# Autodesk Inventor assembly: ThrustBearingAssembly
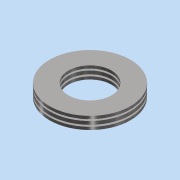
[picture p0: Inventor's stored thumbnail of the model, 180x180]
Saved by Autodesk Inventor 2017 (Build 210142000, 142)
## iProperties
Created: 2016-11-28
Part Number: ThrustBearingAssembly
Document SubType Name: Assembly
Designer: techn
Author: techn
## Documents named in this file (3)
- D:\OneDrive\Documents\Other Projects\Submarine\CAD\midships\BallastSection\ThrustBearing\ThrustBearingAssembly.iam
- D:\OneDrive\Documents\Other Projects\Submarine\CAD\midships\BallastSection\ThrustBearing\NeedleThrustBearing.ipt
- D:\OneDrive\Documents\Other Projects\Submarine\CAD\midships\BallastSection\ThrustBearing\ThrustBearingContactWasher.ipt
## Components (3 placed, 2 different names)
1. NeedleThrustBearing:1 — Mate:1, Tangent:1
2. ThrustBearingContactWasher:1 — Mate:2, Mate:3
3. ThrustBearingContactWasher:2 — Mate:1, Mate:2, Mate:3, Tangent:1
## Relationships (4: Mate 3, Tangent 1)
- Mate:1: NeedleThrustBearing:1 ↔ ThrustBearingContactWasher:2
- Mate:2: ThrustBearingContactWasher:1 ↔ ThrustBearingContactWasher:2
- Mate:3 (1.9844 mm): ThrustBearingContactWasher:1 ↔ ThrustBearingContactWasher:2
- Tangent:1: NeedleThrustBearing:1 ↔ ThrustBearingContactWasher:2
